# Autodesk Inventor assembly: Walls
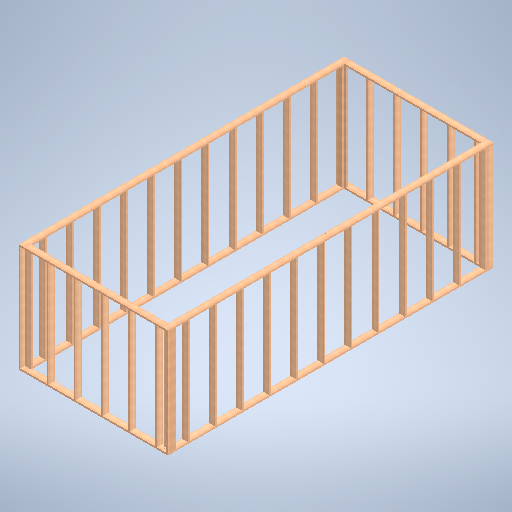
[picture p0: Inventor's stored thumbnail of the model, 512x512]
Saved by Autodesk Inventor 2025 (Build 290162010, 162A)
## iProperties
Created: 2024-09-15
Part Number: Walls
Document SubType Name: Assembly
Designer: Tom
Author: Tom
## Documents named in this file (8)
- C:\Users\Tom\Documents\Inventor\Mobility\Additional_Building\Walls.iam
- C:\Users\Tom\Documents\Inventor\Mobility\Additional_Building\Bottom_Plate_With_Length_144_Inches.ipt
- C:\Users\Tom\Documents\Inventor\Mobility\Additional_Building\Bottom_Plate_With_Length_121_Inches.ipt
- C:\Users\Tom\Documents\Inventor\Mobility\Additional_Building\California_Corner.iam
- C:\Users\Tom\Documents\Inventor\Mobility\Additional_Building\California_Corner_MIR.iam
- C:\Users\Tom\Documents\Inventor\Mobility\Additional_Building\California_Corner_MIR1.iam
- C:\Users\Tom\Documents\Inventor\Mobility\Additional_Building\California_Corner_MIR_MIR.iam
- C:\Users\Tom\Documents\Inventor\Mobility\Additional_Building\Stud.ipt
## Components (48 placed, 7 different names)
1. California_Corner:1 [sub-assembly] — Mate:2, Flush:3, Flush:4
2. California_Corner_MIR:1 [sub-assembly] — Mate:5, Mate:6, Flush:8
3. California_Corner_MIR1:1 [sub-assembly]
4. California_Corner_MIR_MIR:1 [sub-assembly]
5. Bottom_Plate_With_Length_144_Inches:1 — Flush:5
6. Bottom_Plate_With_Length_144_Inches:2
7. Bottom_Plate_With_Length_144_Inches:3 — Mate:1, Flush:1, Flush:2, Mate:4, Flush:6, Flush:8
8. Bottom_Plate_With_Length_144_Inches:4 — Mate:2, Flush:3, Flush:4
9. Bottom_Plate_With_Length_121_Inches:1 — Mate:1, Flush:1, Flush:2, Mate:3, Mate:7
10. Bottom_Plate_With_Length_121_Inches:2
11. Bottom_Plate_With_Length_144_Inches:5
12. Bottom_Plate_With_Length_144_Inches:6
13. Bottom_Plate_With_Length_144_Inches:7
14. Bottom_Plate_With_Length_144_Inches:8
15. Bottom_Plate_With_Length_121_Inches:3 — Flush:7
16. Bottom_Plate_With_Length_121_Inches:4
17. Stud:1 — Mate:4, Flush:6, Mate:5
18. Stud:2
19. Stud:3
20. Stud:4
21. Stud:5
22. Stud:6
23. Stud:7
24. Stud:8
25. Stud:9
26. Stud:10
27. Stud:11
28. Stud:12
29. Stud:13
30. Stud:14
31. Stud:15
32. Stud:16
33. Stud:17
34. Stud:18
35. Stud:19
36. Stud:20
37. Stud:21
38. Stud:22
39. Stud:23 — Flush:7, Mate:6, Mate:7
40. Stud:24
41. Stud:25
42. Stud:26
43. Stud:27
44. Stud:28
45. Stud:29
46. Stud:30
47. Stud:31
48. Stud:32
## Component patterns: (2 elements), (2 elements), (2 elements), (4 elements, first: Bottom_Plate_With_Length_144_Inches:1), (2 elements, first: Bottom_Plate_With_Length_121_Inches:1), Component Pattern 1:2 (4 elements), Component Pattern 2:2 (2 elements), (11 elements, first: Stud:1), Component Pattern 4:2 (11 elements), (5 elements, first: Stud:23), Component Pattern 6:2 (5 elements)
## Relationships (15: Flush 8, Mate 7)
- Mate:1: Bottom_Plate_With_Length_144_Inches:3 ↔ Bottom_Plate_With_Length_121_Inches:1
- Flush:1: Bottom_Plate_With_Length_144_Inches:3 ↔ Bottom_Plate_With_Length_121_Inches:1
- Flush:2: Bottom_Plate_With_Length_144_Inches:3 ↔ Bottom_Plate_With_Length_121_Inches:1
- Mate:2: California_Corner:1 ↔ Bottom_Plate_With_Length_144_Inches:4
- Flush:3: California_Corner:1 ↔ Bottom_Plate_With_Length_144_Inches:4
- Flush:4: California_Corner:1 ↔ Bottom_Plate_With_Length_144_Inches:4
- Flush:5: Bottom_Plate_With_Length_144_Inches:1
- Mate:3 (1536.7 mm): Bottom_Plate_With_Length_121_Inches:1
- Mate:4: Bottom_Plate_With_Length_144_Inches:3 ↔ Stud:1
- Flush:6: Bottom_Plate_With_Length_144_Inches:3 ↔ Stud:1
- Mate:5 (552.45 mm): California_Corner_MIR:1 ↔ Stud:1
- Flush:7: Bottom_Plate_With_Length_121_Inches:3 ↔ Stud:23
- Mate:6 (590.55 mm): California_Corner_MIR:1 ↔ Stud:23
- Mate:7: Bottom_Plate_With_Length_121_Inches:1 ↔ Stud:23
- Flush:8: California_Corner_MIR:1 ↔ Bottom_Plate_With_Length_144_Inches:3
